# Autodesk Inventor assembly: rims
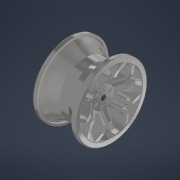
[picture p0: Inventor's stored thumbnail of the model, 180x180]
Saved by Autodesk Inventor 2021.3 (Build 253353000, 353)
## iProperties
Created: 2021-10-18
Part Number: rims
Document SubType Name: Assembly
Designer: ASUS
Author: ASUS
## Documents named in this file (2)
- E:\Inventor\mecanum wheel\rims.iam
- E:\Inventor\31_rim_Mochammad Abdul Aziz.ipt
## Components (1 placed, 1 different names)
1. 31_rim_Mochammad Abdul Aziz:1 — Mate:1, Angle:1
## Relationships (2: Mate 1, Angle 1)
- Mate:1: 31_rim_Mochammad Abdul Aziz:1
- Angle:1 (982 deg): 31_rim_Mochammad Abdul Aziz:1
